# Autodesk Inventor assembly: Mitutoyo-BD-Plan-Apo-system
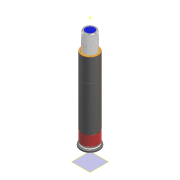
[picture p0: Inventor's stored thumbnail of the model, 180x180]
Saved by Autodesk Inventor 2021 (Build 250183000, 183)
## iProperties
Created: 2022-09-08
Part Number: Mitutoyo-BD-Plan-Apo-system
Document SubType Name: Assembly
Designer: Nikita
Author: Nikita
## Documents named in this file (7)
- C:\Users\Public\GitHub-public\benchtop-hardware\Benchtop\CAD-model-Inventor2021\mesoSPIM\detection_path\Mitutoyo\Mitutoyo-BD-Plan-Apo-system.iam
- C:\Users\Public\GitHub-public\benchtop-hardware\Benchtop\CAD-model-Inventor2021\library\Mitutoyo\BD-Plan-Apo-approx.ipt
- C:\Users\Public\GitHub-public\benchtop-hardware\Benchtop\CAD-model-Inventor2021\library\Thorlabs\accessoires\M2M40S.ipt
- C:\Users\Public\GitHub-public\benchtop-hardware\Benchtop\CAD-model-Inventor2021\library\Thorlabs\lens_tubes\SM2E60.ipt
- C:\Users\Public\GitHub-public\benchtop-hardware\Benchtop\CAD-model-Inventor2021\library\Thorlabs\lens_tubes\SM2L30.ipt
- C:\Users\Public\GitHub-public\benchtop-hardware\Benchtop\CAD-model-Inventor2021\library\Thorlabs\f-mounts\SM2NFM2.ipt
- C:\Users\Public\GitHub-public\benchtop-hardware\Benchtop\custom-parts\detection-accessories\Mitutoyo-Tube-Lens-Objective-assembly\SM2M35-shortened-to-80.7mm.ipt
## Components (6 placed, 6 different names)
1. Mitutoyo-BD-Plan-Apo-approx:1 — Insert:1
2. M2M40S:Adapter — Insert:1, Insert:2, Flush:2
3. SM2L30:ObjFlangeToTubeLens-76.5mm — Insert:2, Insert:3
4. SM2E60:L=150mm — Insert:3, Flush:1, Insert:4, Insert:5
5. SM2NFM2:3 — Insert:4
6. SM2M35-shortened-to-80.7mm:1 — Insert:5
## Relationships (7: Insert 5, Flush 2)
- Insert:1: Mitutoyo-BD-Plan-Apo-approx:1 ↔ M2M40S:Adapter
- Insert:2: M2M40S:Adapter ↔ SM2L30:ObjFlangeToTubeLens-76.5mm
- Insert:3 (0.5 mm): SM2L30:ObjFlangeToTubeLens-76.5mm ↔ SM2E60:L=150mm
- Flush:1 (-10 mm): SM2E60:L=150mm
- Flush:2: M2M40S:Adapter
- Insert:4 (-203.5 mm): SM2E60:L=150mm ↔ SM2NFM2:3
- Insert:5 (0.1 mm): SM2E60:L=150mm ↔ SM2M35-shortened-to-80.7mm:1
